(part 1 of 2)
# Autodesk Inventor assembly: Złożenie całości
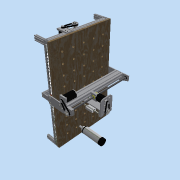
[picture p0: Inventor's stored thumbnail of the model, 180x180]
Saved by Autodesk Inventor 2018 (Build 220112000, 112)
## iProperties
Created: 2019-01-23
Part Number: Złożenie całości
Material: Ogólny
Document SubType Name: Assembly
Designer: Dawid
Author: Dawid
## Documents named in this file (66)
- E:\Frezarka_K2\INVENTOR\ZŁOŻENIA\Złożenie całości.iam
- E:\Frezarka_K2\INVENTOR\RAMA\Profil dolny długi.ipt
- E:\Frezarka_K2\INVENTOR\RAMA\Profil dolny krótki.ipt
- E:\Frezarka_K2\INVENTOR\RAMA\Profil dolny - noga.ipt
- E:\Frezarka_K2\INVENTOR\NAPĘD\Śruba trapezowa 16x4.ipt
- E:\Frezarka_K2\INVENTOR\NAPĘD\Łożysko w obudowie aluminiowej 10mm KP000.ipt
- C:\Users\Dawid\Documents\Inventor\Content Center Files\R2018\pl-PL\DIN 6926\DIN 6926 - M10 x 1,5.ipt
- E:\Frezarka_K2\INVENTOR\NAPĘD\Koło zębate 21 T5 28 2F.ipt
- E:\Frezarka_K2\INVENTOR\NAPĘD\Tuleja zaciskowo rozprężna RCK BK 80 8x15 Clampex.ipt
- C:\Users\Dawid\Documents\Inventor\Content Center Files\R2018\pl-PL\CNS 3932\CNS 3932 - M 4 x 0,7 x 6.ipt
- E:\Frezarka_K2\INVENTOR\NAPĘD\Silnik krokowy SM 60 100-4004AF - 4Nm.ipt
- E:\Frezarka_K2\INVENTOR\NAPĘD\Koło zębate 21 T5 14 2F.ipt
- C:\Users\Dawid\Documents\Inventor\Content Center Files\R2018\pl-PL\CNS 3932\CNS 3932 - M 5 x 0,8 x 12.ipt
- C:\Users\Dawid\Documents\Inventor\Content Center Files\R2018\pl-PL\CNS 3932\CNS 3932 - M 5 x 0,8 x 10.ipt
- E:\Frezarka_K2\INVENTOR\NAPĘD\Nakrętka trapezowa kołnierzowa JFRM-2835TR16x4.ipt
- E:\Frezarka_K2\INVENTOR\NAPĘD\Obudowa nakrętki trapezowej fi 16.ipt
- E:\Frezarka_K2\INVENTOR\RAMA\Profil dolny posuwu osi Y.ipt
- E:\Frezarka_K2\INVENTOR\NAPĘD\Prowadnica liniowa MGN9R 900mm.ipt
- E:\Frezarka_K2\INVENTOR\NAPĘD\Wózek MGN9C.ipt
- C:\Users\Dawid\Documents\Inventor\Content Center Files\R2018\pl-PL\CNS 3932\CNS 3932 - M 3 x 0,5 x 5.ipt
- E:\Frezarka_K2\INVENTOR\WRZECIONA\Wrzeciono Elektrowrzeciono CNC 0.8kw.ipt
- E:\Frezarka_K2\INVENTOR\RAMA\Profil aluminiowy alutec K&K 104080.ipt
- E:\Frezarka_K2\INVENTOR\RAMA\Sklejka stołu.ipt
- E:\Frezarka_K2\INVENTOR\NAPĘD\Prowadnica liniowa typu MGN12H 600mm.ipt
- E:\Frezarka_K2\INVENTOR\NAPĘD\Wózek MGN12H.ipt
- E:\Frezarka_K2\INVENTOR\NAPĘD\Wspornik pionowy osi Z.ipt
- E:\Frezarka_K2\INVENTOR\NAPĘD\Łożysko kulowe jednorzędowe 6200 2RS.ipt
- E:\Frezarka_K2\INVENTOR\NAPĘD\Wspornik pionowy osi Y - lewa strona.ipt
- E:\Frezarka_K2\INVENTOR\NAPĘD\Wspornik pionowy osi Y - prawa strona.ipt
- E:\Frezarka_K2\INVENTOR\NAPĘD\Wspornik łożyska osi Y - prawa strona.ipt
- E:\Frezarka_K2\INVENTOR\NAPĘD\Łożysko kulowe jednorzędowe 3200 2RS.ipt
- E:\Frezarka_K2\INVENTOR\NAPĘD\Śruba trapezowa 16x4 - oś X.ipt
- C:\Users\Dawid\Documents\Inventor\Content Center Files\R2018\pl-PL\CNS 3932\CNS 3932 - M 8 x 1,25 x 14.ipt
- C:\Users\Dawid\Documents\Inventor\Content Center Files\R2018\pl-PL\CNS 3932\CNS 3932 - M 4 x 0,7 x 16.ipt
- E:\Frezarka_K2\INVENTOR\NAPĘD\Uchwyt silnika krokowego osi X - płaski.ipt
- C:\Users\Dawid\Documents\Inventor\Content Center Files\R2018\pl-PL\CNS 3932\CNS 3932 - M 4 x 0,7 x 22.ipt
- E:\Frezarka_K2\INVENTOR\NAPĘD\Pas zębaty 10 T5-305.ipt
- E:\Frezarka_K2\INVENTOR\NAPĘD\Uchwyt łożyska wałka trapezowego osi Y.ipt
- E:\Frezarka_K2\INVENTOR\NAPĘD\Uchwyt łożyska wałka trapezowego osi Y - (blacha łożyska).ipt
- E:\Frezarka_K2\INVENTOR\NAPĘD\Uchwyt silnika krokowego osi Y - płaski.ipt
- E:\Frezarka_K2\INVENTOR\NAPĘD\Łożysko liniowe w obudowie SMAG10UU-L.ipt
- E:\Frezarka_K2\INVENTOR\NAPĘD\Podstawa dolna osi Z.ipt
- E:\Frezarka_K2\INVENTOR\NAPĘD\Pręt liniowy osi Z.ipt
- E:\Frezarka_K2\INVENTOR\NAPĘD\Nakrętka trapezowa kołnierzowa JFRM-2525TR10x3.ipt
- E:\Frezarka_K2\INVENTOR\NAPĘD\Obudowa nakrętki trapezowej fi 10.ipt
- C:\Users\Dawid\Documents\Inventor\Content Center Files\R2018\pl-PL\CNS 3932\CNS 3932 - M 5 x 0,8 x 20.ipt
- E:\Frezarka_K2\INVENTOR\NAPĘD\Śruba trapezowa 10x2 - oś Z.ipt
- E:\Frezarka_K2\INVENTOR\NAPĘD\Silnik krokowy SM 5776-2804MA - 1.89Nm.ipt
- E:\Frezarka_K2\INVENTOR\NAPĘD\Podstawa górna osi Z.ipt
- C:\Users\Dawid\Documents\Inventor\Content Center Files\R2018\pl-PL\CNS 3932\CNS 3932 - M 5 x 0,8 x 25.ipt
- E:\Frezarka_K2\INVENTOR\NAPĘD\Nakrętka trapezowa 10x17.ipt
- C:\Users\Dawid\Documents\Inventor\Content Center Files\R2018\pl-PL\DIN 433-1  A\DIN 433 - 10,5.ipt
- E:\Frezarka_K2\INVENTOR\NAPĘD\Uchwyt górnego łożyska osi Z.ipt
- C:\Users\Dawid\Documents\Inventor\Content Center Files\R2018\pl-PL\CNS 3932\CNS 3932 - M 5 x 0,8 x 22.ipt
- E:\Frezarka_K2\INVENTOR\NAPĘD\Tuleja zaciskowo rozprężna RCK BK 80 10x16 Clampex.ipt
- E:\Frezarka_K2\INVENTOR\NAPĘD\Koło zębate 21 T5 28 2F - toczenie pod tuleję zaciskowo rozprężną fi 10.ipt
- E:\Frezarka_K2\INVENTOR\NAPĘD\Uchwyt silnika krokowego osi Z.ipt
- E:\Frezarka_K2\INVENTOR\NAPĘD\Pas zębaty 10 T5-275.ipt
- C:\Users\Dawid\Documents\Inventor\Content Center Files\R2018\pl-PL\DIN 433-1  A\DIN 433 - 6,4.ipt
- C:\Users\Dawid\Documents\Inventor\Content Center Files\R2018\pl-PL\JIS B 1181 S (1)\JIS B 1181 - A M5.ipt
- C:\Users\Dawid\Documents\Inventor\Content Center Files\R2018\pl-PL\CNS 3932\CNS 3932 - M 5 x 0,8 x 16.ipt
- E:\Frezarka_K2\INVENTOR\NAPĘD\Pas zębaty 10 T5-295.ipt
- C:\Users\Dawid\Documents\Inventor\Content Center Files\R2018\pl-PL\DIN 7991(2)\DIN 7991 - M3x8.ipt
- C:\Users\Dawid\Documents\Inventor\Content Center Files\R2018\pl-PL\DIN 7991(2)\DIN 7991 - M5x12.ipt
- E:\Frezarka_K2\INVENTOR\NAPĘD\Obudowa nakrętki trapezowej fi 16 - oś Y.ipt
- C:\Users\Dawid\Documents\Inventor\Content Center Files\R2018\pl-PL\CNS 3932\CNS 3932 - M 6 x 1 x 30.ipt
## Components (292 placed, 65 different names)
1. Profil dolny długi:1 — Zestawiający:1, Zestawiający:4, Równoległy:19, Równoległy:20, Zestawiający:40, Równoległy:28, Równoległy:29, Zestawiający:41, Równoległy:30, Równoległy:31, Zestawiający:44, Równoległy:36, Równoległy:43, Równoległy:44, Równoległy:45, Zestawiający:65, Równoległy:53
2. Profil dolny krótki:1 — Zestawiający:1, Zestawiający:2, Równoległy:23, Równoległy:24, Zestawiający:38, Równoległy:70
3. Profil dolny długi:2 — Zestawiający:2, Zestawiający:5, Zestawiający:6, Równoległy:21, Równoległy:22, Równoległy:23, Równoległy:24, Zestawiający:39, Równoległy:26, Równoległy:27, Zestawiający:42, Równoległy:32, Równoległy:33, Zestawiający:45, Równoległy:38, Zestawiający:135, Zestawiający:161
4. Profil dolny krótki:2 — Równoległy:19, Równoległy:20, Równoległy:21, Równoległy:22, Równoległy:37, Równoległy:39, Równoległy:52, Zestawiający:135, Zestawiający:172, Zestawiający:176
5. Profil dolny - noga:1 — Zestawiający:5, Zestawiający:42, Równoległy:32, Równoległy:33
6. Profil dolny - noga:2 — Zestawiający:6, Zestawiający:39, Równoległy:26, Równoległy:27
7. Profil dolny - noga:3 — Zestawiający:41, Równoległy:30, Równoległy:31
8. Profil dolny - noga:4 — Zestawiający:4, Zestawiający:40, Równoległy:28, Równoległy:29
9. Śruba trapezowa 16x4:1 — Zestawiający:10, Zestawiający:11, Zestawiający:12, Zestawiający:18, Zestawiający:164, Zestawiający:165, Zestawiający:171, Zestawiający:338, Zestawiający:340
10. Łożysko w obudowie aluminiowej 10mm KP000:2 — Zestawiający:10, Zestawiający:11, Zestawiający:38, Równoległy:70, Zestawiający:161
11. DIN 6926 - zastąpiona przez DIN EN 1663/1666 M10:1 — Zestawiający:12, Zestawiający:169
12. Koło zębate 21 T5 28 2F:1 — Zestawiający:16, Zestawiający:17, Równoległy:72, Zestawiający:178
13. Tuleja zaciskowo rozprężna RCK BK 80 8x15 Clampex:1 — Zestawiający:16, Zestawiający:17, Zestawiający:18, Wstaw:1, Wstaw:2, Wstaw:3, Wstaw:4, Wstaw:5, Wstaw:6, Zestawiający:177
14. CNS 3932 M 4 x 6:1 — Wstaw:1
15. CNS 3932 M 4 x 6:2 — Wstaw:2
16. CNS 3932 M 4 x 6:3 — Wstaw:3
17. CNS 3932 M 4 x 6:4 — Wstaw:4
18. CNS 3932 M 4 x 6:5 — Wstaw:5
19. CNS 3932 M 4 x 6:6 — Wstaw:6
20. Silnik krokowy SM 60 100-4004AF - 4Nm:1 — Zestawiający:21, Zestawiający:22, Wstaw:7, Wstaw:8, Wstaw:9, Wstaw:10, Zestawiający:174, Równoległy:71
21. Koło zębate 21 T5 14 2F:1 — Zestawiający:21, Zestawiający:22, Zestawiający:173, Równoległy:72, Zestawiający:179
22. CNS 3932 M 5 x 12:9 — Wstaw:7
23. CNS 3932 M 5 x 12:2 — Wstaw:8
24. CNS 3932 M 5 x 12:3 — Wstaw:9
25. CNS 3932 M 5 x 12:4 — Wstaw:10
26. Nakrętka trapezowa kołnierzowa JFRM-2835TR16x4:1 — Wstaw:117, Wstaw:118, Wstaw:119, Wstaw:120, Wstaw:121, Wstaw:122, Zestawiający:340, Zestawiający:341
27. Profil dolny posuwu osi Y:1 — Równoległy:40, Zestawiający:77, Równoległy:57, Równoległy:58, Zestawiający:79, Równoległy:60, Równoległy:61, Równoległy:99, Zestawiający:339
28. Prowadnica liniowa MGN9R 900mm:1 — Zestawiający:44, Równoległy:36, Równoległy:37, Zestawiający:50, Zestawiający:51, Zestawiający:52, Zestawiający:53, Wstaw:34, Wstaw:35, Wstaw:36, Wstaw:37, Wstaw:38, Wstaw:39, Wstaw:40, Wstaw:41, Wstaw:42, Wstaw:43, Wstaw:44, Wstaw:45, Wstaw:46, Wstaw:47, Wstaw:48, Wstaw:49, Wstaw:50, Wstaw:51, Wstaw:52
29. Prowadnica liniowa MGN9R 900mm:2 — Zestawiający:45, Równoległy:38, Równoległy:39, Zestawiający:46, Zestawiający:47, Zestawiający:48, Zestawiający:49, Zestawiający:57, Wstaw:15, Wstaw:16, Wstaw:17, Wstaw:18, Wstaw:19, Wstaw:20, Wstaw:21, Wstaw:22, Wstaw:23, Wstaw:24, Wstaw:25, Wstaw:26, Wstaw:27, Wstaw:28, Wstaw:29, Wstaw:30, Wstaw:31, Wstaw:32, Wstaw:33
30. Wózek MGN9C:1 — Zestawiający:46, Zestawiający:47, Zestawiający:80
31. Wózek MGN9C:2 — Zestawiający:48, Zestawiający:49, Zestawiający:57, Zestawiający:81
32. Wózek MGN9C:3 — Zestawiający:50, Zestawiający:51, Zestawiający:82
33. Wózek MGN9C:4 — Zestawiający:52, Zestawiający:53, Równoległy:40, Zestawiający:83
34. CNS 3932 M 3 x 5:1 — Wstaw:15
35. CNS 3932 M 3 x 5:2 — Wstaw:16
36. CNS 3932 M 3 x 5:3 — Wstaw:17
37. CNS 3932 M 3 x 5:4 — Wstaw:18
38. CNS 3932 M 3 x 5:5 — Wstaw:19
39. CNS 3932 M 3 x 5:6 — Wstaw:20
40. CNS 3932 M 3 x 5:7 — Wstaw:21
41. CNS 3932 M 3 x 5:8 — Wstaw:22
42. CNS 3932 M 3 x 5:9 — Wstaw:23
43. CNS 3932 M 3 x 5:10 — Wstaw:24
44. CNS 3932 M 3 x 5:11 — Wstaw:25
45. CNS 3932 M 3 x 5:12 — Wstaw:26
46. CNS 3932 M 3 x 5:13 — Wstaw:27
47. CNS 3932 M 3 x 5:14 — Wstaw:28
48. CNS 3932 M 3 x 5:15 — Wstaw:29
49. CNS 3932 M 3 x 5:16 — Wstaw:30
50. CNS 3932 M 3 x 5:17 — Wstaw:31
51. CNS 3932 M 3 x 5:18 — Wstaw:32
52. CNS 3932 M 3 x 5:19 — Wstaw:33
53. CNS 3932 M 3 x 5:20 — Wstaw:34
54. CNS 3932 M 3 x 5:21 — Wstaw:35
55. CNS 3932 M 3 x 5:22 — Wstaw:36
56. CNS 3932 M 3 x 5:23 — Wstaw:37
57. CNS 3932 M 3 x 5:24 — Wstaw:38
58. CNS 3932 M 3 x 5:25 — Wstaw:39
59. CNS 3932 M 3 x 5:26 — Wstaw:40
60. CNS 3932 M 3 x 5:27 — Wstaw:41
61. CNS 3932 M 3 x 5:28 — Wstaw:42
62. CNS 3932 M 3 x 5:29 — Wstaw:43
63. CNS 3932 M 3 x 5:30 — Wstaw:44
64. CNS 3932 M 3 x 5:31 — Wstaw:45
65. CNS 3932 M 3 x 5:32 — Wstaw:46
66. CNS 3932 M 3 x 5:33 — Wstaw:47
67. CNS 3932 M 3 x 5:34 — Wstaw:48
68. CNS 3932 M 3 x 5:35 — Wstaw:49
69. CNS 3932 M 3 x 5:36 — Wstaw:50
70. CNS 3932 M 3 x 5:37 — Wstaw:51
71. CNS 3932 M 3 x 5:38 — Wstaw:52
72. Wrzeciono Elektrowrzeciono CNC 0.8kw:1 — Zestawiający:94
73. Profil aluminiowy alutec K&K 104080:1 — Zestawiający:66, Równoległy:54, Zestawiający:68, Równoległy:55, Równoległy:63, Równoległy:64, Zestawiający:84, Równoległy:65, Równoległy:66
74. Sklejka stołu:1 — Zestawiający:65, Równoległy:52, Równoległy:53, Zestawiający:94, Zestawiający:170, Zestawiający:175
75. Prowadnica liniowa typu MGN12H 600mm:1 — Zestawiający:68, Równoległy:55, Wstaw:80, Wstaw:81, Wstaw:82, Wstaw:83, Wstaw:84, Wstaw:85, Wstaw:86, Wstaw:87, Wstaw:88, Wstaw:89, Wstaw:90, Wstaw:91, Wstaw:92, Wstaw:93, Wstaw:94, Wstaw:95, Wstaw:96, Wstaw:97, Wstaw:98, Wstaw:99, Wstaw:100, Wstaw:101, Wstaw:102, Zestawiający:72, Zestawiający:73, Równoległy:64
76. Prowadnica liniowa typu MGN12H 600mm:2 — Zestawiający:66, Równoległy:54, Wstaw:57, Wstaw:58, Wstaw:59, Wstaw:60, Wstaw:61, Wstaw:62, Wstaw:63, Wstaw:64, Wstaw:65, Wstaw:66, Wstaw:67, Wstaw:68, Wstaw:69, Wstaw:70, Wstaw:71, Wstaw:72, Wstaw:73, Wstaw:74, Wstaw:75, Wstaw:76, Wstaw:77, Wstaw:78, Wstaw:79, Zestawiający:70, Zestawiający:71, Równoległy:63
77. CNS 3932 M 3 x 5:39 — Wstaw:57
78. CNS 3932 M 3 x 5:40 — Wstaw:58
79. CNS 3932 M 3 x 5:41 — Wstaw:59
80. CNS 3932 M 3 x 5:42 — Wstaw:60
81. CNS 3932 M 3 x 5:43 — Wstaw:61
82. CNS 3932 M 3 x 5:44 — Wstaw:62
83. CNS 3932 M 3 x 5:45 — Wstaw:63
84. CNS 3932 M 3 x 5:46 — Wstaw:64
85. CNS 3932 M 3 x 5:47 — Wstaw:65
86. CNS 3932 M 3 x 5:48 — Wstaw:66
87. CNS 3932 M 3 x 5:49 — Wstaw:67
88. CNS 3932 M 3 x 5:50 — Wstaw:68
89. CNS 3932 M 3 x 5:51 — Wstaw:69
90. CNS 3932 M 3 x 5:52 — Wstaw:70
91. CNS 3932 M 3 x 5:53 — Wstaw:71
92. CNS 3932 M 3 x 5:54 — Wstaw:72
93. CNS 3932 M 3 x 5:55 — Wstaw:73
94. CNS 3932 M 3 x 5:56 — Wstaw:74
95. CNS 3932 M 3 x 5:57 — Wstaw:75
96. CNS 3932 M 3 x 5:58 — Wstaw:76
97. CNS 3932 M 3 x 5:59 — Wstaw:77
98. CNS 3932 M 3 x 5:60 — Wstaw:78
99. CNS 3932 M 3 x 5:61 — Wstaw:79
100. CNS 3932 M 3 x 5:62 — Wstaw:80
101. CNS 3932 M 3 x 5:63 — Wstaw:81
102. CNS 3932 M 3 x 5:64 — Wstaw:82
103. CNS 3932 M 3 x 5:65 — Wstaw:83
104. CNS 3932 M 3 x 5:66 — Wstaw:84
105. CNS 3932 M 3 x 5:67 — Wstaw:85
106. CNS 3932 M 3 x 5:68 — Wstaw:86
107. CNS 3932 M 3 x 5:69 — Wstaw:87
108. CNS 3932 M 3 x 5:70 — Wstaw:88
109. CNS 3932 M 3 x 5:71 — Wstaw:89
110. CNS 3932 M 3 x 5:72 — Wstaw:90
111. CNS 3932 M 3 x 5:73 — Wstaw:91
112. CNS 3932 M 3 x 5:74 — Wstaw:92
113. CNS 3932 M 3 x 5:75 — Wstaw:93
114. CNS 3932 M 3 x 5:76 — Wstaw:94
115. CNS 3932 M 3 x 5:77 — Wstaw:95
116. CNS 3932 M 3 x 5:78 — Wstaw:96
117. CNS 3932 M 3 x 5:79 — Wstaw:97
118. CNS 3932 M 3 x 5:80 — Wstaw:98
119. CNS 3932 M 3 x 5:81 — Wstaw:99
120. CNS 3932 M 3 x 5:82 — Wstaw:100
121. CNS 3932 M 3 x 5:83 — Wstaw:101
122. CNS 3932 M 3 x 5:84 — Wstaw:102
123. Wózek MGN12H:1 — Zestawiający:70, Zestawiający:71, Równoległy:56, Zestawiający:190, Zestawiający:304
124. Wózek MGN12H:2 — Zestawiający:72, Zestawiający:73, Równoległy:56
125. Wspornik pionowy osi Z:1 — Zestawiający:108, Zestawiający:190, Zestawiający:230, Równoległy:85, Wstaw:189, Wstaw:190, Wstaw:191, Wstaw:192, Zestawiający:231, Równoległy:87, Równoległy:89, Zestawiający:243, Zestawiający:265, Zestawiający:304, Równoległy:98, Zestawiający:324, Zestawiający:325, Zestawiający:326, Zestawiający:327, Zestawiający:328, Zestawiający:329, Zestawiający:330, Zestawiający:331, Wstaw:204, Wstaw:205, Wstaw:206, Wstaw:207, Zestawiający:333, Zestawiający:334, Zestawiający:335, Zestawiający:336, Zestawiający:337
126. Łożysko kulowe jednorzędowe 6200 2RS:1 — Zestawiający:78, Równoległy:59, Zestawiający:153, Zestawiający:154
127. Wspornik pionowy osi Y - lewa strona:1 — Zestawiający:77, Równoległy:57, Równoległy:58, Zestawiający:78, Równoległy:59, Zestawiający:80, Zestawiający:81, Wstaw:177, Wstaw:178, Wstaw:200, Wstaw:201
128. Wspornik pionowy osi Y - prawa strona:1 — Zestawiający:79, Równoległy:60, Równoległy:61, Zestawiający:82, Zestawiający:83, Zestawiający:84, Równoległy:65, Równoległy:66, Równoległy:67, Zestawiający:97, Równoległy:68, Zestawiający:120, Wstaw:145, Wstaw:146, Wstaw:147, Wstaw:148, Wstaw:149, Wstaw:150, Wstaw:151, Wstaw:152, Zestawiający:150, Wstaw:179, Wstaw:180, Wstaw:202, Wstaw:203, Zestawiający:316, Zestawiający:317, Zestawiający:318, Zestawiający:319
129. Łożysko kulowe jednorzędowe 3200 2RS:1 — Zestawiający:155, Zestawiający:156
130. Silnik krokowy SM 60 100-4004AF - 4Nm:2 — Zestawiający:118, Zestawiający:119, Zestawiający:120, Wstaw:153, Wstaw:154, Wstaw:155, Wstaw:156, Zestawiający:148
131. Śruba trapezowa 16x4 - oś X:1 — Zestawiający:153, Zestawiający:154, Zestawiający:155, Zestawiający:156, Zestawiający:157, Zestawiający:302
132. Nakrętka trapezowa kołnierzowa JFRM-2835TR16x4:2 — Zestawiający:109, Zestawiający:111, Wstaw:111, Wstaw:112, Wstaw:113, Wstaw:114, Wstaw:115, Wstaw:116, Zestawiający:302
133. Obudowa nakrętki trapezowej fi 16:2 — Zestawiający:108, Zestawiający:109, Zestawiający:111, Zestawiający:222, Zestawiający:333
134. Wspornik łożyska osi Y - prawa strona:1 — Równoległy:67, Zestawiający:97, Równoległy:68, Wstaw:157, Wstaw:158, Wstaw:159, Wstaw:160
135. CNS 3932 M 6 x 30:7 — Wstaw:111
136. CNS 3932 M 6 x 30:8 — Wstaw:112
137. CNS 3932 M 6 x 30:9 — Wstaw:113
138. CNS 3932 M 6 x 30:10 — Wstaw:114
139. CNS 3932 M 6 x 30:11 — Wstaw:115
140. CNS 3932 M 6 x 30:12 — Wstaw:116
141. CNS 3932 M 6 x 30:1 — Wstaw:117
142. CNS 3932 M 6 x 30:2 — Wstaw:118
143. CNS 3932 M 6 x 30:3 — Wstaw:119
144. CNS 3932 M 6 x 30:4 — Wstaw:120
145. CNS 3932 M 6 x 30:5 — Wstaw:121
146. CNS 3932 M 6 x 30:6 — Wstaw:122
147. Koło zębate 21 T5 28 2F:2 — Zestawiający:151, Zestawiający:152, Równoległy:69, Zestawiający:307
148. Tuleja zaciskowo rozprężna RCK BK 80 8x15 Clampex:2 — Wstaw:127, Wstaw:128, Wstaw:129, Wstaw:130, Wstaw:131, Wstaw:132, Zestawiający:151, Zestawiający:152, Zestawiający:157, Zestawiający:305
149. CNS 3932 M 4 x 6:7 — Wstaw:127
150. CNS 3932 M 4 x 6:8 — Wstaw:128
151. CNS 3932 M 4 x 6:9 — Wstaw:129
152. CNS 3932 M 4 x 6:10 — Wstaw:130
153. CNS 3932 M 4 x 6:11 — Wstaw:131
154. CNS 3932 M 4 x 6:12 — Wstaw:132
155. Koło zębate 21 T5 14 2F:2 — Zestawiający:118, Zestawiający:119, Równoległy:69, Zestawiający:306
156. CNS 3932 M 4 x 6:21 — Wstaw:145
157. CNS 3932 M 4 x 6:22 — Wstaw:146
158. CNS 3932 M 4 x 6:23 — Wstaw:147
159. CNS 3932 M 4 x 6:24 — Wstaw:148
160. CNS 3932 M 4 x 6:25 — Wstaw:149
161. CNS 3932 M 4 x 6:26 — Wstaw:150
162. CNS 3932 M 4 x 6:27 — Wstaw:151
163. CNS 3932 M 4 x 6:28 — Wstaw:152
164. CNS 3932 M 5 x 12:10 — Wstaw:153
165. CNS 3932 M 5 x 12:11 — Wstaw:154
166. CNS 3932 M 5 x 12:12 — Wstaw:155, Zestawiający:146
167. CNS 3932 M 5 x 12:13 — Wstaw:156, Zestawiający:147
168. Uchwyt silnika krokowego osi X - płaski:1 — Zestawiający:146, Zestawiający:147, Zestawiający:148, Zestawiający:150, Zestawiający:320, Zestawiający:321, Zestawiający:322, Zestawiający:323
169. CNS 3932 M 4 x 22:1 — Wstaw:157
170. CNS 3932 M 4 x 22:2 — Wstaw:158
171. CNS 3932 M 4 x 22:3 — Wstaw:159
172. CNS 3932 M 4 x 22:4 — Wstaw:160
173. Łożysko kulowe jednorzędowe 3200 2RS:2 — Zestawiający:164, Zestawiający:165, Zestawiający:169
174. Uchwyt łożyska wałka trapezowego osi Y - (blacha łożyska):1
175. Uchwyt łożyska wałka trapezowego osi Y:1 — Zestawiający:170, Zestawiający:171, Zestawiający:172, Wstaw:169, Wstaw:170, Wstaw:171, Wstaw:172, Wstaw:173, Wstaw:174, Wstaw:175, Wstaw:176
176. Uchwyt silnika krokowego osi Y - płaski:1 — Zestawiający:173, Zestawiający:174, Równoległy:71, Zestawiający:175, Zestawiający:176, Wstaw:165, Wstaw:166, Wstaw:167, Wstaw:168
177. Pas zębaty 10 T5-305:2 — Zestawiający:177, Zestawiający:178, Zestawiający:179
178. CNS 3932 M 5 x 10:21 — Wstaw:165
179. CNS 3932 M 5 x 10:22 — Wstaw:166
180. CNS 3932 M 5 x 10:23 — Wstaw:167
181. CNS 3932 M 5 x 10:24 — Wstaw:168
182. CNS 3932 M 4 x 6:29 — Wstaw:169
183. CNS 3932 M 4 x 6:30 — Wstaw:170
184. CNS 3932 M 4 x 6:31 — Wstaw:171
185. CNS 3932 M 4 x 6:32 — Wstaw:172
186. CNS 3932 M 4 x 6:33 — Wstaw:173
187. CNS 3932 M 4 x 6:34 — Wstaw:174
188. CNS 3932 M 4 x 6:35 — Wstaw:175
189. CNS 3932 M 4 x 6:36 — Wstaw:176
190. CNS 3932 M 5 x 10:25 — Wstaw:177
191. CNS 3932 M 5 x 10:26 — Wstaw:178
192. CNS 3932 M 5 x 10:27 — Wstaw:179
193. CNS 3932 M 5 x 10:28 — Wstaw:180
194. Łożysko liniowe w obudowie SMAG10UU-L:1 — Zestawiający:202, Równoległy:75, Równoległy:76, Równoległy:82, Równoległy:92
195. Pręt liniowy osi Z:1 — Zestawiający:201, Równoległy:91, Zestawiający:232
196. Pręt liniowy osi Z:2 — Zestawiający:202, Równoległy:90, Zestawiający:233
197. Łożysko liniowe w obudowie SMAG10UU-L:2 — Zestawiający:201, Równoległy:75, Równoległy:76
198. Nakrętka trapezowa kołnierzowa JFRM-2525TR10x3:1 — Zestawiający:210, Zestawiający:211, Zestawiający:212, Wstaw:181, Wstaw:182, Wstaw:183, Wstaw:184, Wstaw:185, Wstaw:186, Zestawiający:213
199. Obudowa nakrętki trapezowej fi 10:1 — Zestawiający:210, Zestawiający:211, Zestawiający:212, Równoległy:82, Równoległy:92
200. CNS 3932 M 5 x 20:1 — Wstaw:181
201. CNS 3932 M 5 x 20:2 — Wstaw:182
202. CNS 3932 M 5 x 20:3 — Wstaw:183
203. CNS 3932 M 5 x 20:4 — Wstaw:184
204. CNS 3932 M 5 x 20:5 — Wstaw:185
205. CNS 3932 M 5 x 20:6 — Wstaw:186
206. Śruba trapezowa 10x2 - oś Z:1 — Zestawiający:213, Zestawiający:216, Równoległy:81, Zestawiający:229, Zestawiający:234, Zestawiający:236, Zestawiający:237, Zestawiający:240, Zestawiający:250
207. Łożysko kulowe jednorzędowe 6200 2RS:2 — Zestawiający:216, Równoległy:81, Równoległy:88
208. Silnik krokowy SM 5776-2804MA - 1.89Nm:1 — Zestawiający:222, Zestawiający:223, Równoległy:93, Równoległy:95, Zestawiający:265, Zestawiający:270, Zestawiający:275, Zestawiający:278, Zestawiający:279, Zestawiający:280, Zestawiający:291, Zestawiający:293, Zestawiający:295, Zestawiający:303
209. Koło zębate 21 T5 14 2F:3 — Zestawiający:223, Równoległy:93, Równoległy:94, Zestawiający:268, Zestawiający:269
210. Podstawa górna osi Z:1 — Zestawiający:228, Równoległy:84, Zestawiający:230, Równoległy:85, Wstaw:187, Wstaw:188, Równoległy:89, Zestawiający:244, Zestawiający:246, Zestawiający:248, Równoległy:95, Zestawiający:266, Równoległy:96, Równoległy:97
211. Łożysko kulowe jednorzędowe 3200 2RS:3 — Zestawiający:228, Równoległy:84, Zestawiający:229, Zestawiający:238, Zestawiający:241, Zestawiający:245
212. CNS 3932 M 4 x 16:5 — Wstaw:187
213. CNS 3932 M 4 x 16:6 — Wstaw:188
214. CNS 3932 M 5 x 25:1 — Wstaw:189
215. CNS 3932 M 5 x 25:2 — Wstaw:190
216. CNS 3932 M 5 x 25:3 — Wstaw:191
217. CNS 3932 M 5 x 25:4 — Wstaw:192
218. Podstawa dolna osi Z:1 — Zestawiający:231, Równoległy:87, Równoległy:88, Równoległy:90, Równoległy:91, Zestawiający:232, Zestawiający:233, Wstaw:193, Wstaw:194, Równoległy:98
219. CNS 3932 M 4 x 16:7 — Wstaw:193
220. CNS 3932 M 4 x 16:8 — Wstaw:194
221. Nakrętka trapezowa 10x17:1 — Zestawiający:236, Zestawiający:239
222. Nakrętka trapezowa 10x17:2 — Zestawiający:234, Zestawiający:242
223. DIN 433-1 A 10,5:1 — Zestawiający:237, Zestawiający:238, Zestawiający:239
224. DIN 433-1 A 10,5:2 — Zestawiający:240, Zestawiający:241, Zestawiający:242
225. Uchwyt górnego łożyska osi Z:1 — Zestawiający:243, Zestawiający:244, Zestawiający:245, Wstaw:195, Zestawiający:247, Zestawiający:249
226. CNS 3932 M 5 x 22:1 — Wstaw:195
227. CNS 3932 M 5 x 22:15 — Zestawiający:246, Zestawiający:247
228. CNS 3932 M 5 x 22:3 — Zestawiający:248, Zestawiający:249
229. Tuleja zaciskowo rozprężna RCK BK 80 10x16 Clampex:1 — Zestawiający:250, Zestawiający:251, Zestawiający:252, Zestawiający:253, Zestawiający:254, Zestawiający:255, Zestawiający:256, Zestawiający:257, Zestawiający:258, Zestawiający:259, Zestawiający:260, Zestawiający:261, Zestawiający:262, Zestawiający:263, Zestawiający:264
230. Koło zębate 21 T5 28 2F - toczenie pod tuleję zaciskowo rozprężną fi 10:1 — Zestawiający:251, Zestawiający:252, Równoległy:94, Zestawiający:267
231. CNS 3932 M 4 x 6:37 — Zestawiający:253, Zestawiający:254
232. CNS 3932 M 4 x 6:38 — Zestawiający:255, Zestawiający:256
233. CNS 3932 M 4 x 6:39 — Zestawiający:257, Zestawiający:258
234. CNS 3932 M 4 x 6:40 — Zestawiający:259, Zestawiający:260
235. CNS 3932 M 4 x 6:41 — Zestawiający:261, Zestawiający:262
236. CNS 3932 M 4 x 6:42 — Zestawiający:263, Zestawiający:264
237. Uchwyt silnika krokowego osi Z:1 — Zestawiający:266, Równoległy:96, Równoległy:97, Zestawiający:273, Zestawiający:287, Zestawiający:288, Zestawiający:289, Wstaw:196, Wstaw:197, Wstaw:198, Wstaw:199, Zestawiający:303
238. Pas zębaty 10 T5-275:1 — Zestawiający:267, Zestawiający:268, Zestawiający:269
239. CNS 3932 M 5 x 22:4 — Zestawiający:278, Zestawiający:282, Zestawiający:285, Zestawiający:290, Zestawiający:298
240. CNS 3932 M 5 x 22:5 — Zestawiający:279, Zestawiający:283, Zestawiający:286, Zestawiający:294, Zestawiający:296
241. CNS 3932 M 5 x 22:6 — Zestawiający:280, Zestawiający:281, Zestawiający:284, Zestawiający:292, Zestawiający:300
242. CNS 3932 M 5 x 22:7 — Zestawiający:270, Zestawiający:271, Zestawiający:272, Zestawiający:274, Zestawiający:276
243. DIN 433-1 A 6,4:1 — Zestawiający:271, Zestawiający:272, Zestawiający:273
244. DIN 433-1 A 6,4:2 — Zestawiający:274, Zestawiający:275, Zestawiający:277
245. JIS B 1181 Styl 1 - Metryczny A M5:1 — Zestawiający:276, Zestawiający:277
246. DIN 433-1 A 6,4:3 — Zestawiający:281, Zestawiający:284, Zestawiający:288
247. DIN 433-1 A 6,4:4 — Zestawiający:290, Zestawiający:291, Zestawiający:299
248. DIN 433-1 A 6,4:5 — Zestawiający:292, Zestawiający:293, Zestawiający:301
249. DIN 433-1 A 6,4:6 — Zestawiający:282, Zestawiający:285, Zestawiający:289
250. DIN 433-1 A 6,4:7 — Zestawiający:283, Zestawiający:286, Zestawiający:287
251. DIN 433-1 A 6,4:8 — Zestawiający:294, Zestawiający:295, Zestawiający:297
252. JIS B 1181 Styl 1 - Metryczny A M5:2 — Zestawiający:296, Zestawiający:297
253. JIS B 1181 Styl 1 - Metryczny A M5:3 — Zestawiający:298, Zestawiający:299
254. JIS B 1181 Styl 1 - Metryczny A M5:4 — Zestawiający:300, Zestawiający:301
255. CNS 3932 M 5 x 16:1 — Wstaw:196
256. CNS 3932 M 5 x 16:2 — Wstaw:197
257. CNS 3932 M 5 x 16:3 — Wstaw:198
258. CNS 3932 M 5 x 16:4 — Wstaw:199
259. Pas zębaty 10 T5-295:1 — Zestawiający:305, Zestawiający:306, Zestawiający:307
260. CNS 3932 M 8 x 14:1 — Wstaw:200
261. CNS 3932 M 8 x 14:2 — Wstaw:201
262. CNS 3932 M 8 x 14:3 — Wstaw:202
263. CNS 3932 M 8 x 14:4 — Wstaw:203
264. CNS 3932 M 5 x 16:5 — Zestawiający:309, Zestawiający:313, Zestawiający:318
265. CNS 3932 M 5 x 16:6 — Zestawiający:310, Zestawiający:314, Zestawiający:317
266. CNS 3932 M 5 x 16:7 — Zestawiający:311, Zestawiający:315, Zestawiający:316
267. CNS 3932 M 5 x 16:8 — Zestawiający:308, Zestawiający:312, Zestawiający:319
268. DIN 433-1 A 6,4:9 — Zestawiający:309, Zestawiający:313, Zestawiający:322
269. DIN 433-1 A 6,4:10 — Zestawiający:310, Zestawiający:314, Zestawiający:320
270. DIN 433-1 A 6,4:11 — Zestawiający:311, Zestawiający:315, Zestawiający:321
271. DIN 433-1 A 6,4:12 — Zestawiający:308, Zestawiający:312, Zestawiający:323
272. DIN 7991 M3x8:1 — Zestawiający:324
273. DIN 7991 M3x8:2 — Zestawiający:325
274. DIN 7991 M3x8:3 — Zestawiający:326
275. DIN 7991 M3x8:4 — Zestawiający:327
276. DIN 7991 M3x8:5 — Zestawiający:328
277. DIN 7991 M3x8:6 — Zestawiający:329
278. DIN 7991 M3x8:7 — Zestawiający:330
279. DIN 7991 M3x8:8 — Zestawiający:331
280. CNS 3932 M 5 x 20:7 — Wstaw:204
281. CNS 3932 M 5 x 20:8 — Wstaw:205
282. CNS 3932 M 5 x 20:9 — Wstaw:206
283. CNS 3932 M 5 x 20:10 — Wstaw:207
284. DIN 7991 M5x12:2 — Zestawiający:334
285. DIN 7991 M5x12:1 — Zestawiający:335
286. DIN 7991 M5x12:3 — Zestawiający:336
287. DIN 7991 M5x12:4 — Zestawiający:337
288. Obudowa nakrętki trapezowej fi 16 - oś Y:1 — Zestawiający:338, Równoległy:99, Zestawiający:339, Wstaw:208, Wstaw:209, Wstaw:210, Wstaw:211, Zestawiający:341
289. CNS 3932 M 5 x 25:5 — Wstaw:208
290. CNS 3932 M 5 x 25:6 — Wstaw:209
291. CNS 3932 M 5 x 25:7 — Wstaw:210
292. CNS 3932 M 5 x 25:8 — Wstaw:211
## Relationships (436: Mate 200, Insert 175, Flush 61)
- Zestawiający:1 [Mate]: Profil dolny długi:1 ↔ Profil dolny krótki:1
- Zestawiający:2 [Mate]: Profil dolny krótki:1 ↔ Profil dolny długi:2
- Zestawiający:4 [Mate]: Profil dolny długi:1 ↔ Profil dolny - noga:4
- Zestawiający:5 [Mate]: Profil dolny długi:2 ↔ Profil dolny - noga:1
- Zestawiający:6 [Mate]: Profil dolny długi:2 ↔ Profil dolny - noga:2
- Zestawiający:10 [Mate]: Śruba trapezowa 16x4:1 ↔ Łożysko w obudowie aluminiowej 10mm KP000:2
- Zestawiający:11 [Mate] (2 mm): Śruba trapezowa 16x4:1 ↔ Łożysko w obudowie aluminiowej 10mm KP000:2
- Zestawiający:12 [Mate]: Śruba trapezowa 16x4:1 ↔ DIN 6926 - zastąpiona przez DIN EN 1663/1666 M10:1
- Zestawiający:16 [Mate]: Koło zębate 21 T5 28 2F:1 ↔ Tuleja zaciskowo rozprężna RCK BK 80 8x15 Clampex:1
- Zestawiający:17 [Mate]: Koło zębate 21 T5 28 2F:1 ↔ Tuleja zaciskowo rozprężna RCK BK 80 8x15 Clampex:1
- Zestawiający:18 [Mate]: Śruba trapezowa 16x4:1 ↔ Tuleja zaciskowo rozprężna RCK BK 80 8x15 Clampex:1
- Wstaw:1 [Insert]: Tuleja zaciskowo rozprężna RCK BK 80 8x15 Clampex:1 ↔ CNS 3932 M 4 x 6:1
- Wstaw:2 [Insert]: Tuleja zaciskowo rozprężna RCK BK 80 8x15 Clampex:1 ↔ CNS 3932 M 4 x 6:2
- Wstaw:3 [Insert]: Tuleja zaciskowo rozprężna RCK BK 80 8x15 Clampex:1 ↔ CNS 3932 M 4 x 6:3
- Wstaw:4 [Insert]: Tuleja zaciskowo rozprężna RCK BK 80 8x15 Clampex:1 ↔ CNS 3932 M 4 x 6:4
- Wstaw:5 [Insert]: Tuleja zaciskowo rozprężna RCK BK 80 8x15 Clampex:1 ↔ CNS 3932 M 4 x 6:5
- Wstaw:6 [Insert]: Tuleja zaciskowo rozprężna RCK BK 80 8x15 Clampex:1 ↔ CNS 3932 M 4 x 6:6
- Zestawiający:21 [Mate]: Silnik krokowy SM 60 100-4004AF - 4Nm:1 ↔ Koło zębate 21 T5 14 2F:1
- Zestawiający:22 [Mate] (1 mm): Silnik krokowy SM 60 100-4004AF - 4Nm:1 ↔ Koło zębate 21 T5 14 2F:1
- Wstaw:7 [Insert]: Silnik krokowy SM 60 100-4004AF - 4Nm:1 ↔ CNS 3932 M 5 x 12:9
- Wstaw:8 [Insert]: Silnik krokowy SM 60 100-4004AF - 4Nm:1 ↔ CNS 3932 M 5 x 12:2
- Wstaw:9 [Insert]: Silnik krokowy SM 60 100-4004AF - 4Nm:1 ↔ CNS 3932 M 5 x 12:3
- Wstaw:10 [Insert]: Silnik krokowy SM 60 100-4004AF - 4Nm:1 ↔ CNS 3932 M 5 x 12:4
- Równoległy:19 [Flush]: Profil dolny długi:1 ↔ Profil dolny krótki:2
- Równoległy:20 [Flush]: Profil dolny długi:1 ↔ Profil dolny krótki:2
- Równoległy:21 [Flush]: Profil dolny długi:2 ↔ Profil dolny krótki:2
- Równoległy:22 [Flush]: Profil dolny długi:2 ↔ Profil dolny krótki:2
- Równoległy:23 [Flush]: Profil dolny krótki:1 ↔ Profil dolny długi:2
- Równoległy:24 [Flush]: Profil dolny krótki:1 ↔ Profil dolny długi:2
- Zestawiający:38 [Mate]: Profil dolny krótki:1 ↔ Łożysko w obudowie aluminiowej 10mm KP000:2
- Zestawiający:39 [Mate]: Profil dolny długi:2 ↔ Profil dolny - noga:2
- Równoległy:26 [Flush]: Profil dolny długi:2 ↔ Profil dolny - noga:2
- Równoległy:27 [Flush]: Profil dolny długi:2 ↔ Profil dolny - noga:2
- Zestawiający:40 [Mate]: Profil dolny długi:1 ↔ Profil dolny - noga:4
- Równoległy:28 [Flush]: Profil dolny długi:1 ↔ Profil dolny - noga:4
- Równoległy:29 [Flush]: Profil dolny długi:1 ↔ Profil dolny - noga:4
- Zestawiający:41 [Mate]: Profil dolny długi:1 ↔ Profil dolny - noga:3
- Równoległy:30 [Flush]: Profil dolny długi:1 ↔ Profil dolny - noga:3
- Równoległy:31 [Flush]: Profil dolny długi:1 ↔ Profil dolny - noga:3
- Zestawiający:42 [Mate]: Profil dolny długi:2 ↔ Profil dolny - noga:1
- Równoległy:32 [Flush]: Profil dolny długi:2 ↔ Profil dolny - noga:1
- Równoległy:33 [Flush]: Profil dolny długi:2 ↔ Profil dolny - noga:1
- Zestawiający:44 [Mate]: Profil dolny długi:1 ↔ Prowadnica liniowa MGN9R 900mm:1
- Równoległy:36 [Flush] (25.5 mm): Profil dolny długi:1 ↔ Prowadnica liniowa MGN9R 900mm:1
- Równoległy:37 [Flush] (25 mm): Profil dolny krótki:2 ↔ Prowadnica liniowa MGN9R 900mm:1
- Zestawiający:45 [Mate]: Profil dolny długi:2 ↔ Prowadnica liniowa MGN9R 900mm:2
- Równoległy:38 [Flush] (25.5 mm): Profil dolny długi:2 ↔ Prowadnica liniowa MGN9R 900mm:2
- Równoległy:39 [Flush] (25 mm): Profil dolny krótki:2 ↔ Prowadnica liniowa MGN9R 900mm:2
- Zestawiający:46 [Mate]: Prowadnica liniowa MGN9R 900mm:2 ↔ Wózek MGN9C:1
- Zestawiający:47 [Mate]: Prowadnica liniowa MGN9R 900mm:2 ↔ Wózek MGN9C:1
- Zestawiający:48 [Mate]: Prowadnica liniowa MGN9R 900mm:2 ↔ Wózek MGN9C:2
- Zestawiający:49 [Mate]: Prowadnica liniowa MGN9R 900mm:2 ↔ Wózek MGN9C:2
- Zestawiający:50 [Mate]: Prowadnica liniowa MGN9R 900mm:1 ↔ Wózek MGN9C:3
- Zestawiający:51 [Mate]: Prowadnica liniowa MGN9R 900mm:1 ↔ Wózek MGN9C:3
- Zestawiający:52 [Mate]: Prowadnica liniowa MGN9R 900mm:1 ↔ Wózek MGN9C:4
- Zestawiający:53 [Mate]: Prowadnica liniowa MGN9R 900mm:1 ↔ Wózek MGN9C:4
- Równoległy:40 [Flush]: Profil dolny posuwu osi Y:1 ↔ Wózek MGN9C:4
- Równoległy:43 [Flush]: Profil dolny długi:1
- Równoległy:44 [Flush]: Profil dolny długi:1
- Równoległy:45 [Flush]: Profil dolny długi:1
- Zestawiający:57 [Mate]: Prowadnica liniowa MGN9R 900mm:2 ↔ Wózek MGN9C:2
- Wstaw:15 [Insert]: Prowadnica liniowa MGN9R 900mm:2 ↔ CNS 3932 M 3 x 5:1
- Wstaw:16 [Insert]: Prowadnica liniowa MGN9R 900mm:2 ↔ CNS 3932 M 3 x 5:2
- Wstaw:17 [Insert]: Prowadnica liniowa MGN9R 900mm:2 ↔ CNS 3932 M 3 x 5:3
- Wstaw:18 [Insert]: Prowadnica liniowa MGN9R 900mm:2 ↔ CNS 3932 M 3 x 5:4
- Wstaw:19 [Insert]: Prowadnica liniowa MGN9R 900mm:2 ↔ CNS 3932 M 3 x 5:5
- Wstaw:20 [Insert]: Prowadnica liniowa MGN9R 900mm:2 ↔ CNS 3932 M 3 x 5:6
- Wstaw:21 [Insert]: Prowadnica liniowa MGN9R 900mm:2 ↔ CNS 3932 M 3 x 5:7
- Wstaw:22 [Insert]: Prowadnica liniowa MGN9R 900mm:2 ↔ CNS 3932 M 3 x 5:8
- Wstaw:23 [Insert]: Prowadnica liniowa MGN9R 900mm:2 ↔ CNS 3932 M 3 x 5:9
- Wstaw:24 [Insert]: Prowadnica liniowa MGN9R 900mm:2 ↔ CNS 3932 M 3 x 5:10
- Wstaw:25 [Insert]: Prowadnica liniowa MGN9R 900mm:2 ↔ CNS 3932 M 3 x 5:11
- Wstaw:26 [Insert]: Prowadnica liniowa MGN9R 900mm:2 ↔ CNS 3932 M 3 x 5:12
- Wstaw:27 [Insert]: Prowadnica liniowa MGN9R 900mm:2 ↔ CNS 3932 M 3 x 5:13
- Wstaw:28 [Insert]: Prowadnica liniowa MGN9R 900mm:2 ↔ CNS 3932 M 3 x 5:14
- Wstaw:29 [Insert]: Prowadnica liniowa MGN9R 900mm:2 ↔ CNS 3932 M 3 x 5:15
- Wstaw:30 [Insert]: Prowadnica liniowa MGN9R 900mm:2 ↔ CNS 3932 M 3 x 5:16
- Wstaw:31 [Insert]: Prowadnica liniowa MGN9R 900mm:2 ↔ CNS 3932 M 3 x 5:17
- Wstaw:32 [Insert]: Prowadnica liniowa MGN9R 900mm:2 ↔ CNS 3932 M 3 x 5:18
- Wstaw:33 [Insert]: Prowadnica liniowa MGN9R 900mm:2 ↔ CNS 3932 M 3 x 5:19
- Wstaw:34 [Insert]: Prowadnica liniowa MGN9R 900mm:1 ↔ CNS 3932 M 3 x 5:20
- Wstaw:35 [Insert]: Prowadnica liniowa MGN9R 900mm:1 ↔ CNS 3932 M 3 x 5:21
- Wstaw:36 [Insert]: Prowadnica liniowa MGN9R 900mm:1 ↔ CNS 3932 M 3 x 5:22
- Wstaw:37 [Insert]: Prowadnica liniowa MGN9R 900mm:1 ↔ CNS 3932 M 3 x 5:23
- Wstaw:38 [Insert]: Prowadnica liniowa MGN9R 900mm:1 ↔ CNS 3932 M 3 x 5:24
- Wstaw:39 [Insert]: Prowadnica liniowa MGN9R 900mm:1 ↔ CNS 3932 M 3 x 5:25
- Wstaw:40 [Insert]: Prowadnica liniowa MGN9R 900mm:1 ↔ CNS 3932 M 3 x 5:26
- Wstaw:41 [Insert]: Prowadnica liniowa MGN9R 900mm:1 ↔ CNS 3932 M 3 x 5:27
- Wstaw:42 [Insert]: Prowadnica liniowa MGN9R 900mm:1 ↔ CNS 3932 M 3 x 5:28
- Wstaw:43 [Insert]: Prowadnica liniowa MGN9R 900mm:1 ↔ CNS 3932 M 3 x 5:29
- Wstaw:44 [Insert]: Prowadnica liniowa MGN9R 900mm:1 ↔ CNS 3932 M 3 x 5:30
- Wstaw:45 [Insert]: Prowadnica liniowa MGN9R 900mm:1 ↔ CNS 3932 M 3 x 5:31
- Wstaw:46 [Insert]: Prowadnica liniowa MGN9R 900mm:1 ↔ CNS 3932 M 3 x 5:32
- Wstaw:47 [Insert]: Prowadnica liniowa MGN9R 900mm:1 ↔ CNS 3932 M 3 x 5:33
- Wstaw:48 [Insert]: Prowadnica liniowa MGN9R 900mm:1 ↔ CNS 3932 M 3 x 5:34
- Wstaw:49 [Insert]: Prowadnica liniowa MGN9R 900mm:1 ↔ CNS 3932 M 3 x 5:35
- Wstaw:50 [Insert]: Prowadnica liniowa MGN9R 900mm:1 ↔ CNS 3932 M 3 x 5:36
- Wstaw:51 [Insert]: Prowadnica liniowa MGN9R 900mm:1 ↔ CNS 3932 M 3 x 5:37
- Wstaw:52 [Insert]: Prowadnica liniowa MGN9R 900mm:1 ↔ CNS 3932 M 3 x 5:38
- Zestawiający:65 [Mate]: Profil dolny długi:1 ↔ Sklejka stołu:1
- Równoległy:52 [Flush]: Profil dolny krótki:2 ↔ Sklejka stołu:1
- Równoległy:53 [Flush]: Profil dolny długi:1 ↔ Sklejka stołu:1
- Zestawiający:66 [Mate]: Profil aluminiowy alutec K&K 104080:1 ↔ Prowadnica liniowa typu MGN12H 600mm:2
- Równoległy:54 [Flush] (14 mm): Profil aluminiowy alutec K&K 104080:1 ↔ Prowadnica liniowa typu MGN12H 600mm:2
- Zestawiający:68 [Mate]: Profil aluminiowy alutec K&K 104080:1 ↔ Prowadnica liniowa typu MGN12H 600mm:1
- Równoległy:55 [Flush] (14 mm): Profil aluminiowy alutec K&K 104080:1 ↔ Prowadnica liniowa typu MGN12H 600mm:1
- Wstaw:57 [Insert]: Prowadnica liniowa typu MGN12H 600mm:2 ↔ CNS 3932 M 3 x 5:39
- Wstaw:58 [Insert]: Prowadnica liniowa typu MGN12H 600mm:2 ↔ CNS 3932 M 3 x 5:40
- Wstaw:59 [Insert]: Prowadnica liniowa typu MGN12H 600mm:2 ↔ CNS 3932 M 3 x 5:41
- Wstaw:60 [Insert]: Prowadnica liniowa typu MGN12H 600mm:2 ↔ CNS 3932 M 3 x 5:42
- Wstaw:61 [Insert]: Prowadnica liniowa typu MGN12H 600mm:2 ↔ CNS 3932 M 3 x 5:43
- Wstaw:62 [Insert]: Prowadnica liniowa typu MGN12H 600mm:2 ↔ CNS 3932 M 3 x 5:44
- Wstaw:63 [Insert]: Prowadnica liniowa typu MGN12H 600mm:2 ↔ CNS 3932 M 3 x 5:45
- Wstaw:64 [Insert]: Prowadnica liniowa typu MGN12H 600mm:2 ↔ CNS 3932 M 3 x 5:46
- Wstaw:65 [Insert]: Prowadnica liniowa typu MGN12H 600mm:2 ↔ CNS 3932 M 3 x 5:47
- Wstaw:66 [Insert]: Prowadnica liniowa typu MGN12H 600mm:2 ↔ CNS 3932 M 3 x 5:48
- Wstaw:67 [Insert]: Prowadnica liniowa typu MGN12H 600mm:2 ↔ CNS 3932 M 3 x 5:49
- Wstaw:68 [Insert]: Prowadnica liniowa typu MGN12H 600mm:2 ↔ CNS 3932 M 3 x 5:50
- Wstaw:69 [Insert]: Prowadnica liniowa typu MGN12H 600mm:2 ↔ CNS 3932 M 3 x 5:51
- Wstaw:70 [Insert]: Prowadnica liniowa typu MGN12H 600mm:2 ↔ CNS 3932 M 3 x 5:52
- Wstaw:71 [Insert]: Prowadnica liniowa typu MGN12H 600mm:2 ↔ CNS 3932 M 3 x 5:53
- Wstaw:72 [Insert]: Prowadnica liniowa typu MGN12H 600mm:2 ↔ CNS 3932 M 3 x 5:54
- Wstaw:73 [Insert]: Prowadnica liniowa typu MGN12H 600mm:2 ↔ CNS 3932 M 3 x 5:55
- Wstaw:74 [Insert]: Prowadnica liniowa typu MGN12H 600mm:2 ↔ CNS 3932 M 3 x 5:56
- Wstaw:75 [Insert]: Prowadnica liniowa typu MGN12H 600mm:2 ↔ CNS 3932 M 3 x 5:57
- Wstaw:76 [Insert]: Prowadnica liniowa typu MGN12H 600mm:2 ↔ CNS 3932 M 3 x 5:58
- Wstaw:77 [Insert]: Prowadnica liniowa typu MGN12H 600mm:2 ↔ CNS 3932 M 3 x 5:59
- Wstaw:78 [Insert]: Prowadnica liniowa typu MGN12H 600mm:2 ↔ CNS 3932 M 3 x 5:60
- Wstaw:79 [Insert]: Prowadnica liniowa typu MGN12H 600mm:2 ↔ CNS 3932 M 3 x 5:61
- Wstaw:80 [Insert]: Prowadnica liniowa typu MGN12H 600mm:1 ↔ CNS 3932 M 3 x 5:62
- Wstaw:81 [Insert]: Prowadnica liniowa typu MGN12H 600mm:1 ↔ CNS 3932 M 3 x 5:63
- Wstaw:82 [Insert]: Prowadnica liniowa typu MGN12H 600mm:1 ↔ CNS 3932 M 3 x 5:64
- Wstaw:83 [Insert]: Prowadnica liniowa typu MGN12H 600mm:1 ↔ CNS 3932 M 3 x 5:65
- Wstaw:84 [Insert]: Prowadnica liniowa typu MGN12H 600mm:1 ↔ CNS 3932 M 3 x 5:66
- Wstaw:85 [Insert]: Prowadnica liniowa typu MGN12H 600mm:1 ↔ CNS 3932 M 3 x 5:67
- Wstaw:86 [Insert]: Prowadnica liniowa typu MGN12H 600mm:1 ↔ CNS 3932 M 3 x 5:68
- Wstaw:87 [Insert]: Prowadnica liniowa typu MGN12H 600mm:1 ↔ CNS 3932 M 3 x 5:69
- Wstaw:88 [Insert]: Prowadnica liniowa typu MGN12H 600mm:1 ↔ CNS 3932 M 3 x 5:70
- Wstaw:89 [Insert]: Prowadnica liniowa typu MGN12H 600mm:1 ↔ CNS 3932 M 3 x 5:71
- Wstaw:90 [Insert]: Prowadnica liniowa typu MGN12H 600mm:1 ↔ CNS 3932 M 3 x 5:72
- Wstaw:91 [Insert]: Prowadnica liniowa typu MGN12H 600mm:1 ↔ CNS 3932 M 3 x 5:73
- Wstaw:92 [Insert]: Prowadnica liniowa typu MGN12H 600mm:1 ↔ CNS 3932 M 3 x 5:74